# Autodesk Inventor assembly: Assembly1
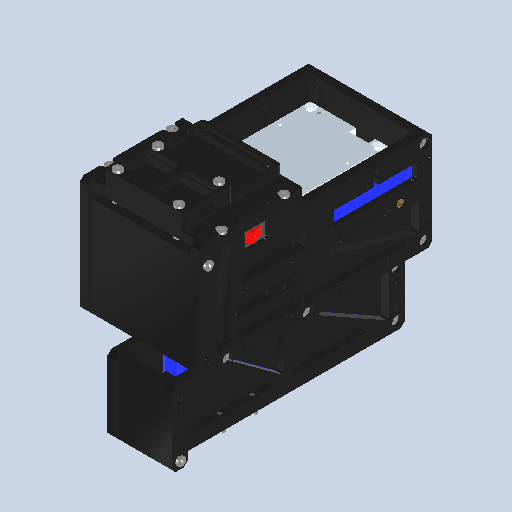
[picture p0: Inventor's stored thumbnail of the model, 512x512]
Saved by Autodesk Inventor 2022.4 (Build 264492000, 492)
## iProperties
Created: 2021-04-12
Part Number: Assembly1
Document SubType Name: Assembly
Designer: masato
Mass: 620.128 g
Surface Area: 2948.67 cm^2
Volume: 396.034 cm^3
Density: 1.56585 g/cm^3
Author: masato
## Documents named in this file (28)
- C:\Users\supra\Documents\GitHub\OpenPlatform_ver3_0\UpperBody\Cockpit\Cockpit.iam
- C:\Users\supra\Documents\GitHub\OpenPlatform_ver3_0\Ready_Made\Auvidea_J120\Auvidea_J120.ipt
- C:\Users\supra\Documents\GitHub\OpenPlatform_ver3_0\Ready_Made\Jetson_TX2\Jetson_TX2.ipt
- C:\Users\supra\Documents\GitHub\OpenPlatform_ver3_0\UpperBody\Cockpit\Cockpit_upper_side_frame.ipt
- C:\Users\supra\Documents\GitHub\OpenPlatform_ver3_0\UpperBody\Cockpit\Cockpit_upper_side_frame_MIR.ipt
- C:\Users\supra\Documents\GitHub\OpenPlatform_ver3_0\UpperBody\Cockpit\Cockpit_upper_front_frame.ipt
- C:\Users\supra\Documents\GitHub\OpenPlatform_ver3_0\Ready_Made\KCD11-A-101011BB.ipt
- C:\Users\supra\Documents\GitHub\OpenPlatform_ver3_0\UpperBody\Cockpit\Cockpit_upper_middle_frame.ipt
- C:\Users\supra\Documents\GitHub\OpenPlatform_ver3_0\UpperBody\Cockpit\Cockpit_upper_bottom_frame.ipt
- C:\Users\supra\Documents\GitHub\OpenPlatform_ver3_0\UpperBody\Cockpit\Cockpit_lower_side_frame.ipt
- C:\Users\supra\Documents\GitHub\OpenPlatform_ver3_0\UpperBody\Cockpit\Cockpit_lower_side_frame_MIR.ipt
- C:\Users\supra\Documents\GitHub\OpenPlatform_ver3_0\UpperBody\Cockpit\Cockpit_lower_front_frame.ipt
- C:\Users\supra\Documents\GitHub\OpenPlatform_ver3_0\UpperBody\Cockpit\Cockpit_lower_bottom_frame.ipt
- C:\Users\supra\Documents\GitHub\OpenPlatform_ver3_0\UpperBody\Cockpit\Cockpit_upper_top_frame.ipt
- C:\Users\supra\Documents\GitHub\OpenPlatform_ver3_0\UpperBody\Cockpit\Cockpit_lower_back_door.ipt
- C:\Users\supra\Documents\GitHub\OpenPlatform_ver3_0\UpperBody\Cockpit\MainBoard_cover.ipt
- C:\Users\supra\Documents\GitHub\OpenPlatform_ver3_0\Ready_Made\HP-G570-2600S3.ipt
- C:\Users\supra\Documents\GitHub\OpenPlatform_ver3_0\UpperBody\Cockpit\J120_cover.ipt
- C:\Users\supra\Documents\GitHub\OpenPlatform_ver3_0\Ready_Made\Screw\M3-6.ipt
- C:\Users\supra\Documents\GitHub\OpenPlatform_ver3_0\Ready_Made\Screw\M3-8.ipt
- C:\Users\supra\Documents\GitHub\OpenPlatform_ver3_0\Ready_Made\Screw\M3-10.ipt
- C:\Users\supra\Documents\GitHub\OpenPlatform_ver3_0\Ready_Made\UD-43040.ipt
- C:\Users\supra\Documents\GitHub\OpenPlatform_ver3_0\UpperBody\Cockpit\StartStopSwitch_lower_cover.ipt
- C:\Users\supra\Documents\GitHub\OpenPlatform_ver3_0\UpperBody\Cockpit\StartStopSwitch_upper_cover.ipt
- C:\Users\supra\Documents\GitHub\OpenPlatform_ver3_0\UpperBody\Cockpit\Voltmeter_lower_cover.ipt
- C:\Users\supra\Documents\GitHub\OpenPlatform_ver3_0\Ready_Made\Neodymium_magnet_Phi3_T3.ipt
- C:\Users\supra\Documents\GitHub\OpenPlatform_ver3_0\Ready_Made\Antenna.ipt
- C:\Users\supra\Documents\GitHub\OpenPlatform_ver3_0\UpperBody\Cockpit\Cockpit_upper_back_door.ipt
## Components (98 placed, 27 different names)
1. Auvidea_J120:1 — 挿入:52, 挿入:55, 挿入:90, 挿入:91
2. Jetson_TX2:1 — 挿入:52, 挿入:55
3. KCD11-A-101011BB:1 — メイト:2, メイト:3, メイト:4
4. KCD11-A-101011BB:2 — メイト:13, メイト:14, メイト:15
5. Cockpit_upper_middle_frame:1 — フラッシュ:1, メイト:8, メイト:9, 挿入:92, 挿入:93, 挿入:130, 挿入:131, 挿入:132, 挿入:133
6. Cockpit_upper_bottom_frame:1 — 挿入:67, 挿入:73, 挿入:87, 挿入:88, 挿入:94, 挿入:120, 挿入:121, 挿入:122, 挿入:123, 挿入:160
7. Cockpit_lower_bottom_frame:1 — 挿入:74, 挿入:75, メイト:17, 挿入:103, 挿入:104, 挿入:105, 挿入:106
8. Cockpit_upper_side_frame:1 — メイト:2, メイト:3, メイト:4, フラッシュ:1, メイト:8, メイト:9, メイト:12, 挿入:67, 挿入:94, 挿入:97, 挿入:115, 挿入:116, 挿入:117, 挿入:118, 挿入:128, 挿入:156, 挿入:157, メイト:20, メイト:24, メイト:25, 挿入:175, 角度:2, 挿入:180, 挿入:192, 挿入:193
9. Cockpit_upper_side_frame_MIR:1 — メイト:13, メイト:14, メイト:15, 挿入:96, 挿入:110, 挿入:111, 挿入:112, 挿入:113, 挿入:129, メイト:21, メイト:22, メイト:23, 挿入:174, 挿入:176, 挿入:181, 挿入:190, 挿入:191
10. Cockpit_upper_front_frame:1 — 挿入:156, 挿入:157, 挿入:174, メイト:26
11. Cockpit_lower_side_frame:1 — 挿入:74, 挿入:100, 挿入:101, 挿入:158, 角度:1, 挿入:165, 挿入:166, 挿入:167, 挿入:177, 挿入:179
12. Cockpit_lower_side_frame_MIR:1 — 挿入:73, 挿入:75, メイト:18, 挿入:107, 挿入:108, 挿入:159, 挿入:160, 挿入:162, 挿入:163, 挿入:164, 挿入:178
13. Cockpit_lower_front_frame:1 — メイト:19, 挿入:158, 挿入:159
14. Cockpit_upper_top_frame:1 — 挿入:96, 挿入:97, 挿入:134, 挿入:135, 挿入:136, 挿入:137, 挿入:140, 挿入:141, 挿入:142, 挿入:143, 挿入:144, 挿入:145, 挿入:150, 挿入:151, 挿入:152, 挿入:153, 挿入:154, 挿入:155
15. MainBoard_cover:1 — 挿入:87, 挿入:88, 挿入:124, 挿入:125, 挿入:126, 挿入:127
16. HP-G570-2600S3:1 — メイト:17, メイト:18, メイト:19
17. Cockpit_lower_back_door:1 — 角度:1, 挿入:168, 挿入:169, 挿入:170, 挿入:171, 挿入:172, 挿入:173, 挿入:177
18. J120_cover:1 — 挿入:90, 挿入:91, 挿入:92, 挿入:93
19. M3-6:1 — 挿入:101
20. M3-6:2 — 挿入:100
21. M3-6:4 — 挿入:103
22. M3-6:5 — 挿入:104
23. M3-6:6 — 挿入:107
24. M3-6:8 — 挿入:108
25. M3-6:9 — 挿入:106
26. M3-6:10 — 挿入:105
27. M3-6:11 — 挿入:110
28. M3-6:12 — 挿入:111
29. M3-6:13 — 挿入:112
30. M3-6:14 — 挿入:113
31. M3-6:16 — 挿入:116
32. M3-6:17 — 挿入:117
33. M3-6:18 — 挿入:118
34. M3-6:20 — 挿入:115
35. M3-8:1 — 挿入:120
36. M3-8:2 — 挿入:121
37. M3-8:3 — 挿入:122
38. M3-8:4 — 挿入:123
39. M3-10:1 — 挿入:124
40. M3-10:2 — 挿入:125
41. M3-10:3 — 挿入:126
42. M3-10:4 — 挿入:127
43. UD-43040:1 — 挿入:128
44. UD-43040:2 — 挿入:129
45. M3-10:5 — 挿入:130
46. M3-10:6 — 挿入:131
47. M3-10:7 — 挿入:133
48. M3-10:8 — 挿入:132
49. M3-6:21 — 挿入:134
50. M3-6:22 — 挿入:135
51. M3-6:23 — 挿入:137
52. M3-6:24 — 挿入:136
53. StartStopSwitch_lower_cover:1 — 挿入:138, 挿入:139, 挿入:140, 挿入:141
54. StartStopSwitch_upper_cover:1 — 挿入:138, 挿入:139, 挿入:146, 挿入:147, 挿入:148, 挿入:149
55. M3-8:5 — 挿入:142
56. M3-8:6 — 挿入:143
57. M3-8:7 — 挿入:144
58. M3-8:8 — 挿入:145
59. M3-6:25 — 挿入:146
60. M3-6:26 — 挿入:147
61. M3-6:27 — 挿入:148
62. M3-6:28 — 挿入:149
63. Voltmeter_lower_cover:1 — 挿入:150, 挿入:151
64. M3-8:9 — 挿入:152
65. M3-8:10 — 挿入:155
66. M3-8:11 — 挿入:154
67. M3-8:12 — 挿入:153
68. Neodymium_magnet_Phi3_T3:1 — 挿入:162
69. Neodymium_magnet_Phi3_T3:2 — 挿入:163
70. Neodymium_magnet_Phi3_T3:3 — 挿入:164
71. Neodymium_magnet_Phi3_T3:4 — 挿入:171
72. Neodymium_magnet_Phi3_T3:5 — 挿入:172
73. Neodymium_magnet_Phi3_T3:6 — 挿入:173
74. Neodymium_magnet_Phi3_T3:7 — 挿入:168
75. Neodymium_magnet_Phi3_T3:8 — 挿入:169
76. Neodymium_magnet_Phi3_T3:9 — 挿入:170
77. Neodymium_magnet_Phi3_T3:10 — 挿入:165
78. Neodymium_magnet_Phi3_T3:11 — 挿入:166
79. Neodymium_magnet_Phi3_T3:12 — 挿入:167
80. Antenna:1 — メイト:20, メイト:24, メイト:25
81. Antenna:2 — メイト:21, メイト:22, メイト:23
82. Cockpit_upper_back_door:1 — 挿入:175, 挿入:176, 角度:2, 挿入:186, 挿入:187, 挿入:188, 挿入:189
83. UD-43040:3 — 挿入:180, 挿入:185
84. UD-43040:4 — 挿入:181, 挿入:183
85. UD-43040:5 — 挿入:179, 挿入:184
86. UD-43040:6 — 挿入:178, 挿入:182
87. M3-8:13 — 挿入:183
88. M3-8:14 — 挿入:182
89. M3-8:15 — 挿入:185
90. M3-8:16 — 挿入:184
91. Neodymium_magnet_Phi3_T3:13 — 挿入:188
92. Neodymium_magnet_Phi3_T3:14 — 挿入:187
93. Neodymium_magnet_Phi3_T3:15 — 挿入:186
94. Neodymium_magnet_Phi3_T3:16 — 挿入:192
95. Neodymium_magnet_Phi3_T3:17 — 挿入:189
96. Neodymium_magnet_Phi3_T3:18 — 挿入:190
97. Neodymium_magnet_Phi3_T3:19 — 挿入:191
98. Neodymium_magnet_Phi3_T3:20 — 挿入:193
## Relationships (126: Insert 104, Mate 19, Angle 2, Flush 1)
- 挿入:52 [Insert] (7 mm): Auvidea_J120:1 ↔ Jetson_TX2:1
- 挿入:55 [Insert] (7 mm): Auvidea_J120:1 ↔ Jetson_TX2:1
- メイト:2 [Mate]: KCD11-A-101011BB:1 ↔ Cockpit_upper_side_frame:1
- メイト:3 [Mate] (0.05 mm): KCD11-A-101011BB:1 ↔ Cockpit_upper_side_frame:1
- メイト:4 [Mate] (0.05 mm): KCD11-A-101011BB:1 ↔ Cockpit_upper_side_frame:1
- フラッシュ:1 [Flush]: Cockpit_upper_middle_frame:1 ↔ Cockpit_upper_side_frame:1
- メイト:8 [Mate] (0.025 mm): Cockpit_upper_middle_frame:1 ↔ Cockpit_upper_side_frame:1
- メイト:9 [Mate] (0.025 mm): Cockpit_upper_middle_frame:1 ↔ Cockpit_upper_side_frame:1
- メイト:12 [Mate]: Cockpit_upper_side_frame:1
- メイト:13 [Mate]: KCD11-A-101011BB:2 ↔ Cockpit_upper_side_frame_MIR:1
- メイト:14 [Mate] (0.05 mm): KCD11-A-101011BB:2 ↔ Cockpit_upper_side_frame_MIR:1
- メイト:15 [Mate] (0.05 mm): KCD11-A-101011BB:2 ↔ Cockpit_upper_side_frame_MIR:1
- 挿入:67 [Insert]: Cockpit_upper_bottom_frame:1 ↔ Cockpit_upper_side_frame:1
- 挿入:73 [Insert]: Cockpit_upper_bottom_frame:1 ↔ Cockpit_lower_side_frame_MIR:1
- 挿入:74 [Insert]: Cockpit_lower_bottom_frame:1 ↔ Cockpit_lower_side_frame:1
- 挿入:75 [Insert]: Cockpit_lower_bottom_frame:1 ↔ Cockpit_lower_side_frame_MIR:1
- メイト:17 [Mate]: Cockpit_lower_bottom_frame:1 ↔ HP-G570-2600S3:1
- メイト:18 [Mate]: Cockpit_lower_side_frame_MIR:1 ↔ HP-G570-2600S3:1
- メイト:19 [Mate]: Cockpit_lower_front_frame:1 ↔ HP-G570-2600S3:1
- 挿入:87 [Insert]: Cockpit_upper_bottom_frame:1 ↔ MainBoard_cover:1
- 挿入:88 [Insert]: Cockpit_upper_bottom_frame:1 ↔ MainBoard_cover:1
- 挿入:90 [Insert]: Auvidea_J120:1 ↔ J120_cover:1
- 挿入:91 [Insert]: Auvidea_J120:1 ↔ J120_cover:1
- 挿入:92 [Insert]: Cockpit_upper_middle_frame:1 ↔ J120_cover:1
- 挿入:93 [Insert]: Cockpit_upper_middle_frame:1 ↔ J120_cover:1
- 挿入:94 [Insert]: Cockpit_upper_bottom_frame:1 ↔ Cockpit_upper_side_frame:1
- 挿入:96 [Insert]: Cockpit_upper_side_frame_MIR:1 ↔ Cockpit_upper_top_frame:1
- 挿入:97 [Insert]: Cockpit_upper_side_frame:1 ↔ Cockpit_upper_top_frame:1
- 挿入:100 [Insert]: Cockpit_lower_side_frame:1 ↔ M3-6:2
- 挿入:101 [Insert]: Cockpit_lower_side_frame:1 ↔ M3-6:1
- 挿入:103 [Insert]: Cockpit_lower_bottom_frame:1 ↔ M3-6:4
- 挿入:104 [Insert]: Cockpit_lower_bottom_frame:1 ↔ M3-6:5
- 挿入:105 [Insert]: Cockpit_lower_bottom_frame:1 ↔ M3-6:10
- 挿入:106 [Insert]: Cockpit_lower_bottom_frame:1 ↔ M3-6:9
- 挿入:107 [Insert]: Cockpit_lower_side_frame_MIR:1 ↔ M3-6:6
- 挿入:108 [Insert]: Cockpit_lower_side_frame_MIR:1 ↔ M3-6:8
- 挿入:110 [Insert]: Cockpit_upper_side_frame_MIR:1 ↔ M3-6:11
- 挿入:111 [Insert]: Cockpit_upper_side_frame_MIR:1 ↔ M3-6:12
- 挿入:112 [Insert]: Cockpit_upper_side_frame_MIR:1 ↔ M3-6:13
- 挿入:113 [Insert]: Cockpit_upper_side_frame_MIR:1 ↔ M3-6:14
- 挿入:115 [Insert]: Cockpit_upper_side_frame:1 ↔ M3-6:20
- 挿入:116 [Insert]: Cockpit_upper_side_frame:1 ↔ M3-6:16
- 挿入:117 [Insert]: Cockpit_upper_side_frame:1 ↔ M3-6:17
- 挿入:118 [Insert]: Cockpit_upper_side_frame:1 ↔ M3-6:18
- 挿入:120 [Insert]: Cockpit_upper_bottom_frame:1 ↔ M3-8:1
- 挿入:121 [Insert]: Cockpit_upper_bottom_frame:1 ↔ M3-8:2
- 挿入:122 [Insert]: Cockpit_upper_bottom_frame:1 ↔ M3-8:3
- 挿入:123 [Insert]: Cockpit_upper_bottom_frame:1 ↔ M3-8:4
- 挿入:124 [Insert]: MainBoard_cover:1 ↔ M3-10:1
- 挿入:125 [Insert]: MainBoard_cover:1 ↔ M3-10:2
- 挿入:126 [Insert]: MainBoard_cover:1 ↔ M3-10:3
- 挿入:127 [Insert]: MainBoard_cover:1 ↔ M3-10:4
- 挿入:128 [Insert]: Cockpit_upper_side_frame:1 ↔ UD-43040:1
- 挿入:129 [Insert]: Cockpit_upper_side_frame_MIR:1 ↔ UD-43040:2
- 挿入:130 [Insert]: Cockpit_upper_middle_frame:1 ↔ M3-10:5
- 挿入:131 [Insert]: Cockpit_upper_middle_frame:1 ↔ M3-10:6
- 挿入:132 [Insert]: Cockpit_upper_middle_frame:1 ↔ M3-10:8
- 挿入:133 [Insert]: Cockpit_upper_middle_frame:1 ↔ M3-10:7
- 挿入:134 [Insert]: Cockpit_upper_top_frame:1 ↔ M3-6:21
- 挿入:135 [Insert]: Cockpit_upper_top_frame:1 ↔ M3-6:22
- 挿入:136 [Insert]: Cockpit_upper_top_frame:1 ↔ M3-6:24
- 挿入:137 [Insert]: Cockpit_upper_top_frame:1 ↔ M3-6:23
- 挿入:138 [Insert]: StartStopSwitch_lower_cover:1 ↔ StartStopSwitch_upper_cover:1
- 挿入:139 [Insert]: StartStopSwitch_lower_cover:1 ↔ StartStopSwitch_upper_cover:1
- 挿入:140 [Insert]: Cockpit_upper_top_frame:1 ↔ StartStopSwitch_lower_cover:1
- 挿入:141 [Insert]: Cockpit_upper_top_frame:1 ↔ StartStopSwitch_lower_cover:1
- 挿入:142 [Insert]: Cockpit_upper_top_frame:1 ↔ M3-8:5
- 挿入:143 [Insert]: Cockpit_upper_top_frame:1 ↔ M3-8:6
- 挿入:144 [Insert]: Cockpit_upper_top_frame:1 ↔ M3-8:7
- 挿入:145 [Insert]: Cockpit_upper_top_frame:1 ↔ M3-8:8
- 挿入:146 [Insert]: StartStopSwitch_upper_cover:1 ↔ M3-6:25
- 挿入:147 [Insert]: StartStopSwitch_upper_cover:1 ↔ M3-6:26
- 挿入:148 [Insert]: StartStopSwitch_upper_cover:1 ↔ M3-6:27
- 挿入:149 [Insert]: StartStopSwitch_upper_cover:1 ↔ M3-6:28
- 挿入:150 [Insert]: Cockpit_upper_top_frame:1 ↔ Voltmeter_lower_cover:1
- 挿入:151 [Insert]: Cockpit_upper_top_frame:1 ↔ Voltmeter_lower_cover:1
- 挿入:152 [Insert]: Cockpit_upper_top_frame:1 ↔ M3-8:9
- 挿入:153 [Insert]: Cockpit_upper_top_frame:1 ↔ M3-8:12
- 挿入:154 [Insert]: Cockpit_upper_top_frame:1 ↔ M3-8:11
- 挿入:155 [Insert]: Cockpit_upper_top_frame:1 ↔ M3-8:10
- 挿入:156 [Insert]: Cockpit_upper_side_frame:1 ↔ Cockpit_upper_front_frame:1
- 挿入:157 [Insert]: Cockpit_upper_side_frame:1 ↔ Cockpit_upper_front_frame:1
- 挿入:158 [Insert]: Cockpit_lower_side_frame:1 ↔ Cockpit_lower_front_frame:1
- 挿入:159 [Insert]: Cockpit_lower_side_frame_MIR:1 ↔ Cockpit_lower_front_frame:1
- 角度:1 [Angle] (0 deg): Cockpit_lower_side_frame:1 ↔ Cockpit_lower_back_door:1
- 挿入:160 [Insert]: Cockpit_upper_bottom_frame:1 ↔ Cockpit_lower_side_frame_MIR:1
- 挿入:162 [Insert]: Cockpit_lower_side_frame_MIR:1 ↔ Neodymium_magnet_Phi3_T3:1
- 挿入:163 [Insert]: Cockpit_lower_side_frame_MIR:1 ↔ Neodymium_magnet_Phi3_T3:2
- 挿入:164 [Insert]: Cockpit_lower_side_frame_MIR:1 ↔ Neodymium_magnet_Phi3_T3:3
- 挿入:165 [Insert]: Cockpit_lower_side_frame:1 ↔ Neodymium_magnet_Phi3_T3:10
- 挿入:166 [Insert]: Cockpit_lower_side_frame:1 ↔ Neodymium_magnet_Phi3_T3:11
- 挿入:167 [Insert]: Cockpit_lower_side_frame:1 ↔ Neodymium_magnet_Phi3_T3:12
- 挿入:168 [Insert]: Cockpit_lower_back_door:1 ↔ Neodymium_magnet_Phi3_T3:7
- 挿入:169 [Insert]: Cockpit_lower_back_door:1 ↔ Neodymium_magnet_Phi3_T3:8
- 挿入:170 [Insert]: Cockpit_lower_back_door:1 ↔ Neodymium_magnet_Phi3_T3:9
- 挿入:171 [Insert]: Cockpit_lower_back_door:1 ↔ Neodymium_magnet_Phi3_T3:4
- 挿入:172 [Insert]: Cockpit_lower_back_door:1 ↔ Neodymium_magnet_Phi3_T3:5
- 挿入:173 [Insert]: Cockpit_lower_back_door:1 ↔ Neodymium_magnet_Phi3_T3:6
- メイト:20 [Mate]: Cockpit_upper_side_frame:1 ↔ Antenna:1
- メイト:21 [Mate]: Cockpit_upper_side_frame_MIR:1 ↔ Antenna:2
- メイト:22 [Mate] (0.25 mm): Cockpit_upper_side_frame_MIR:1 ↔ Antenna:2
- メイト:23 [Mate] (0.25 mm): Cockpit_upper_side_frame_MIR:1 ↔ Antenna:2
- メイト:24 [Mate] (0.25 mm): Cockpit_upper_side_frame:1 ↔ Antenna:1
- メイト:25 [Mate] (0.25 mm): Cockpit_upper_side_frame:1 ↔ Antenna:1
- 挿入:174 [Insert]: Cockpit_upper_side_frame_MIR:1 ↔ Cockpit_upper_front_frame:1
- メイト:26 [Mate]: Cockpit_upper_front_frame:1
- 挿入:175 [Insert]: Cockpit_upper_side_frame:1 ↔ Cockpit_upper_back_door:1
- 挿入:176 [Insert]: Cockpit_upper_side_frame_MIR:1 ↔ Cockpit_upper_back_door:1
- 角度:2 [Angle] (0 deg): Cockpit_upper_side_frame:1 ↔ Cockpit_upper_back_door:1
- 挿入:177 [Insert]: Cockpit_lower_side_frame:1 ↔ Cockpit_lower_back_door:1
- 挿入:178 [Insert]: Cockpit_lower_side_frame_MIR:1 ↔ UD-43040:6
- 挿入:179 [Insert]: Cockpit_lower_side_frame:1 ↔ UD-43040:5
- 挿入:180 [Insert]: Cockpit_upper_side_frame:1 ↔ UD-43040:3
- 挿入:181 [Insert]: Cockpit_upper_side_frame_MIR:1 ↔ UD-43040:4
- 挿入:182 [Insert]: UD-43040:6 ↔ M3-8:14
- 挿入:183 [Insert]: UD-43040:4 ↔ M3-8:13
- 挿入:184 [Insert]: UD-43040:5 ↔ M3-8:16
- 挿入:185 [Insert]: UD-43040:3 ↔ M3-8:15
- 挿入:186 [Insert]: Cockpit_upper_back_door:1 ↔ Neodymium_magnet_Phi3_T3:15
- 挿入:187 [Insert]: Cockpit_upper_back_door:1 ↔ Neodymium_magnet_Phi3_T3:14
- 挿入:188 [Insert]: Cockpit_upper_back_door:1 ↔ Neodymium_magnet_Phi3_T3:13
- 挿入:189 [Insert]: Cockpit_upper_back_door:1 ↔ Neodymium_magnet_Phi3_T3:17
- 挿入:190 [Insert]: Cockpit_upper_side_frame_MIR:1 ↔ Neodymium_magnet_Phi3_T3:18
- 挿入:191 [Insert]: Cockpit_upper_side_frame_MIR:1 ↔ Neodymium_magnet_Phi3_T3:19
- 挿入:192 [Insert]: Cockpit_upper_side_frame:1 ↔ Neodymium_magnet_Phi3_T3:16
- 挿入:193 [Insert]: Cockpit_upper_side_frame:1 ↔ Neodymium_magnet_Phi3_T3:20
